# Autodesk Inventor assembly: Frank
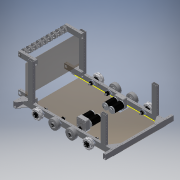
[picture p0: Inventor's stored thumbnail of the model, 180x180]
Saved by Autodesk Inventor 2018 (Build 220112000, 112)
## iProperties
Created: 2018-09-06
Part Number: Frank
Document SubType Name: Assembly
Designer: baoan
Author: baoan
## Documents named in this file (6)
- C:\Users\baoan\Documents\Inventor\Bunnybots\Frank.iam
- C:\Users\baoan\Documents\Inventor\Bunnybots\Drivetrain\Drivetrain.iam
- C:\Users\baoan\Documents\Inventor\Bunnybots\Electrical_board\Belly_pan.ipt
- C:\Users\baoan\Documents\Inventor\Bunnybots\Intake&Outake\Intake&Outake.iam
- C:\Users\baoan\Documents\Inventor\Bunnybots\Intake&Outake\Intake_backboard.ipt
- C:\Users\baoan\Documents\Inventor\Bunnybots\Intake&Outake\Outtake_vertical_frame.ipt
## Components (6 placed, 5 different names)
1. Drivetrain:1 [sub-assembly] — Mate:1, Mate:2, Mate:3, Mate:4, Flush:1, Mate:5, Mate:8, Flush:3, Mate:9, Mate:10, Flush:4, Mate:11
2. Belly_pan:1 — Mate:1, Mate:2, Mate:3
3. Intake&Outake:1 [sub-assembly] — Mate:4, Flush:1, Mate:5, Mate:6, Flush:2, Mate:7
4. Intake_backboard:1 — Mate:6, Flush:2, Mate:7
5. Outtake_vertical_frame:1 — Mate:8, Flush:3, Mate:9
6. Outtake_vertical_frame:2 — Mate:10, Flush:4, Mate:11
## Relationships (15: Mate 11, Flush 4)
- Mate:1: Drivetrain:1 ↔ Belly_pan:1
- Mate:2: Drivetrain:1 ↔ Belly_pan:1
- Mate:3: Drivetrain:1 ↔ Belly_pan:1
- Mate:4: Drivetrain:1 ↔ Intake&Outake:1
- Flush:1: Drivetrain:1 ↔ Intake&Outake:1
- Mate:5: Drivetrain:1 ↔ Intake&Outake:1
- Mate:6 (25.4 mm): Intake&Outake:1 ↔ Intake_backboard:1
- Flush:2: Intake&Outake:1 ↔ Intake_backboard:1
- Mate:7: Intake&Outake:1 ↔ Intake_backboard:1
- Mate:8: Drivetrain:1 ↔ Outtake_vertical_frame:1
- Flush:3: Drivetrain:1 ↔ Outtake_vertical_frame:1
- Mate:9: Drivetrain:1 ↔ Outtake_vertical_frame:1
- Mate:10: Drivetrain:1 ↔ Outtake_vertical_frame:2
- Flush:4: Drivetrain:1 ↔ Outtake_vertical_frame:2
- Mate:11: Drivetrain:1 ↔ Outtake_vertical_frame:2
